# Autodesk Inventor assembly: lazysusan3
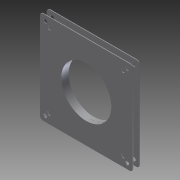
[picture p0: Inventor's stored thumbnail of the model, 180x180]
Saved by Autodesk Inventor 2011 (Build 150239000, 239)
## iProperties
Created: 2011-09-17
Part Number: lazysusan3
Document SubType Name: Assembly
Designer: Matthew
Author: Matthew
## Documents named in this file (3)
- C:\Users\Matthew\Documents\matthew_autocad\prlite\lazy susan\lazysusan3.iam
- C:\Users\Matthew\Documents\matthew_autocad\prlite\lazy susan\3.ipt
- C:\Users\Matthew\Documents\matthew_autocad\prlite\lazy susan\4.ipt
## Components (2 placed, 2 different names)
1. 3:1 — Mate:1, Mate:2
2. 4:1 — Mate:1, Mate:2
## Relationships (2: Mate 2)
- Mate:1: 3:1 ↔ 4:1
- Mate:2: 3:1 ↔ 4:1
